# Autodesk Inventor assembly: Assembly6
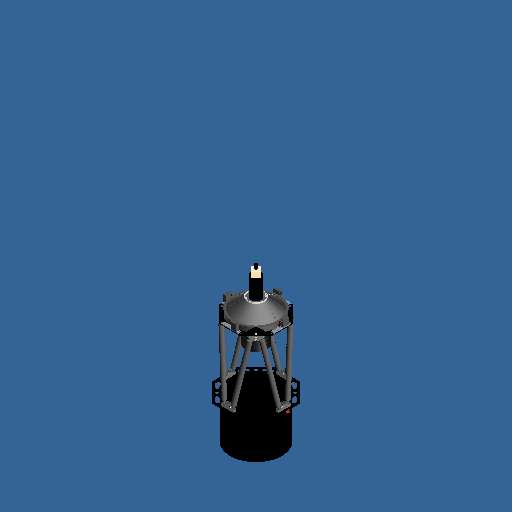
[picture p0: Inventor's stored thumbnail of the model, 512x512]
Saved by Autodesk Inventor 2026.2 (Build 302298000, 298)
## iProperties
Created: 2025-12-09
Part Number: Assembly6
Document SubType Name: Assembly
Designer: Thoma
Mass: 27295.5 g
Surface Area: 25498 cm^2
Volume: 10830.6 cm^3
Density: 2.52023 g/cm^3
Author: Thoma
## Documents named in this file (21)
- C:\Users\Thoma\OneDrive\Desktop\dir\telescope_cover\main\version_2\Main_v4.iam
- C:\Users\Thoma\OneDrive\Desktop\dir\telescope_cover\telescope\version_3\Telescope_End.ipt
- C:\Users\Thoma\OneDrive\Desktop\dir\telescope_cover\telescope\version_3\Triangle.ipt
- C:\Users\Thoma\OneDrive\Desktop\dir\telescope_cover\telescope\version_3\Triangle_Bracket_Top.ipt
- C:\Users\Thoma\OneDrive\Desktop\dir\telescope_cover\telescope\version_3\Carbon_Fibre.ipt
- C:\Users\Thoma\OneDrive\Desktop\dir\telescope_cover\telescope\version_3\5mm Screw.ipt
- C:\Users\Thoma\OneDrive\Desktop\dir\telescope_cover\telescope\version_3\35mm_bolt.ipt
- C:\Users\Thoma\OneDrive\Desktop\dir\telescope_cover\telescope\version_3\Triangle_Bracket_Bottom_MIR.ipt
- C:\Users\Thoma\OneDrive\Desktop\dir\telescope_cover\telescope\version_3\Telescope_Base.ipt
- C:\Users\Thoma\OneDrive\Desktop\dir\telescope_cover\telescope\version_3\Full_shaft_Simplify_3.ipt
- C:\Users\Thoma\OneDrive\Desktop\dir\telescope_cover\cover\Conic_Cover_Simplify_1.ipt
- C:\Users\Thoma\OneDrive\Desktop\dir\telescope_cover\telescope\version_3\30mm_bolt.ipt
- C:\Users\Thoma\OneDrive\Desktop\dir\telescope_cover\telescope\version_3\Baffle.ipt
- C:\Users\Thoma\OneDrive\Desktop\dir\telescope_cover\telescope\version_3\Bottom_End_Top.ipt
- C:\Users\Thoma\OneDrive\Desktop\dir\telescope_cover\cover\Cover_Lower_v3.ipt
- C:\Users\Thoma\OneDrive\Desktop\dir\telescope_cover\cover\Cover_Upper_v3.ipt
- C:\Users\Thoma\OneDrive\Desktop\dir\telescope_cover\telescope\version_3\4mm_0.5_Screw.ipt
- C:\Users\Thoma\OneDrive\Desktop\dir\telescope_cover\cover\Base_Plate_v2.ipt
- C:\Users\Thoma\OneDrive\Desktop\dir\telescope_cover\servo\motor_basic.ipt
- C:\Users\Thoma\OneDrive\Desktop\dir\telescope_cover\cover\rod_v6.ipt
- C:\Users\Thoma\OneDrive\Desktop\dir\telescope_cover\telescope\version_3\Laser.ipt
## Components (80 placed, 20 different names)
1. motor_basic:3 — Mate:174, Flush:138, Flush:176, Mate:175, Mate:176, Angle:85
2. motor_basic:2 — Mate:163, Flush:136, Mate:166, Mate:167, Flush:137, Angle:87
3. motor_basic:4 — Mate:191, Flush:177, Flush:178, Mate:216, Mate:219, Angle:86
4. motor_basic:5 — Mate:192, Flush:179, Flush:180, Mate:193, Mate:204, Angle:83
5. Laser:1 — Mate:215, Flush:218, Flush:219
6. Laser:2 — Mate:214, Flush:220, Flush:221
7. rod_v6:4 — Mate:216, Mate:217, Mate:218, Mate:219, Tangent:23, Angle:86
8. Full_shaft_Simplify_3:1 — Tangent:24, Tangent:25
9. Full_shaft_Simplify_3:2 — Tangent:26
10. Full_shaft_Simplify_3:3 — Tangent:27
11. Full_shaft_Simplify_3:4 — Tangent:28
12. Full_shaft_Simplify_3:5 — Tangent:29
13. Full_shaft_Simplify_3:6 — Tangent:30
14. Full_shaft_Simplify_3:7 — Tangent:32
15. Full_shaft_Simplify_3:8 — Tangent:31, Tangent:33
16. Baffle:1 — Mate:83
17. Carbon_Fibre:1 — Mate:7, Mate:11, Flush:1, Mate:12, Mate:13, Mate:14, Mate:15, Mate:62, Flush:2, Flush:3, Flush:4, Flush:5, Mate:83, Mate:92, Mate:93, Mate:96, Mate:97, Mate:98, Mate:99, Mate:100, Mate:123, Mate:124, Mate:125, Mate:213
18. Telescope_Base:1 — Mate:62, Angle:31, Mate:89, Mate:90, Angle:40, Mate:108, Mate:109, Angle:48, Mate:110, Mate:111, Angle:49, Mate:112, Mate:113, Angle:50, Mate:214, Mate:215, Flush:218, Flush:221
19. Telescope_End:1 — Mate:1, Mate:2, Angle:2, Mate:7, Mate:54, Mate:55, Angle:26, Angle:31, Mate:86, Mate:88, Mate:91, Angle:41, Mate:101, Angle:45, Angle:46, Mate:114, Mate:115, Angle:51, Mate:116, Mate:117, Angle:52, Mate:118, Mate:119, Angle:53, Mate:141, Mate:142, Mate:143, Mate:158, Mate:159, Mate:160, Mate:185, Mate:186, Mate:187, Mate:188, Mate:189, Mate:190
20. Triangle_Bracket_Top:5 — Mate:116, Mate:117, Angle:52, Mate:129, Flush:110, Angle:60
21. Triangle_Bracket_Top:4 — Mate:101, Angle:45, Angle:46, Mate:104, Mate:105, Mate:106, Flush:103, Angle:47
22. Triangle_Bracket_Top:3 — Mate:86, Mate:88, Mate:94, Angle:54, Angle:55, Mate:122, Flush:106, Angle:56
23. Triangle_Bracket_Top:1 — Mate:1, Mate:2, Angle:2, Mate:8, Mate:9, Angle:4, Mate:47, Angle:22, Mate:58
24. Triangle:1 — Mate:8, Mate:9, Angle:4, Mate:11, Flush:1, Angle:5, Angle:6, Mate:46, Mate:70, Mate:71
25. Triangle:5 — Mate:92, Mate:93, Mate:94, Mate:102, Mate:128, Flush:109, Angle:59, Mate:132, Flush:181, Angle:81
26. Triangle:6 — Mate:96, Mate:97, Mate:98, Flush:101, Angle:43, Flush:102, Angle:44, Mate:103, Mate:104, Mate:105, Mate:107
27. Triangle:7 — Mate:123, Mate:124, Mate:125, Mate:126, Flush:107, Angle:57, Mate:127, Flush:108, Angle:58, Mate:130, Mate:131
28. 35mm_bolt:6 — Mate:122, Flush:106, Angle:56
29. 35mm_bolt:7 — Mate:129, Flush:110, Angle:60
30. 35mm_bolt:4 — Mate:46, Mate:47, Angle:22
31. 35mm_bolt:5 — Mate:106, Flush:103, Angle:47
32. 5mm Screw:9 — Mate:100, Flush:102, Angle:44
33. 5mm Screw:13 — Mate:213, Flush:181, Angle:81
34. 5mm Screw:8 — Mate:99, Flush:101, Angle:43
35. 5mm Screw:10 — Mate:126, Flush:107, Angle:57
36. 5mm Screw:2 — Mate:14, Mate:15, Angle:6
37. 5mm Screw:1 — Mate:12, Mate:13, Angle:5
38. 5mm Screw:11 — Mate:127, Flush:108, Angle:58
39. 5mm Screw:12 — Mate:128, Flush:109, Angle:59
40. 30mm_bolt:7 — Mate:120, Flush:104, Angle:54
41. 30mm_bolt:1 — Mate:121, Flush:105, Angle:55
42. 30mm_bolt:8 — Mate:80, Flush:13, Angle:39
43. 30mm_bolt:6 — Mate:78, Flush:11, Angle:37
44. 30mm_bolt:3 — Mate:79, Flush:12, Angle:38
45. 30mm_bolt:2 — Mate:77, Flush:10, Angle:36
46. Triangle_Bracket_Bottom_MIR:4 — Mate:118, Mate:119, Angle:53, Tangent:24
47. Triangle_Bracket_Bottom_MIR:3 — Mate:114, Mate:115, Angle:51, Mate:120, Flush:104, Mate:121, Flush:105, Tangent:27, Tangent:28
48. Triangle_Bracket_Bottom_MIR:2 — Mate:55, Mate:58, Angle:26, Mate:77, Flush:10, Angle:36, Mate:78, Flush:11, Angle:37, Tangent:30, Tangent:31
49. Triangle_Bracket_Bottom_MIR:1 — Mate:54, Mate:79, Flush:12, Angle:38, Mate:80, Flush:13, Angle:39, Mate:91, Angle:41, Tangent:29, Tangent:32
50. Bottom_End_Top:4 — Mate:112, Mate:113, Angle:50, Tangent:26, Tangent:33
51. Bottom_End_Top:3 — Mate:110, Mate:111, Angle:49, Flush:219, Tangent:25
52. Bottom_End_Top:2 — Mate:108, Mate:109, Angle:48
53. Bottom_End_Top:1 — Mate:89, Mate:90, Angle:40, Flush:220
54. Conic_Cover_Simplify_1:1 — Flush:2, Mate:131, Mate:132
55. Conic_Cover_Simplify_1:2 — Flush:3, Mate:102, Mate:103
56. Conic_Cover_Simplify_1:3 — Flush:4, Mate:70, Mate:107
57. Conic_Cover_Simplify_1:4 — Mate:71, Flush:5, Mate:130
58. Cover_Lower_v3:2 — Tangent:22, Mate:205, Mate:206, Mate:207, Mate:208, Mate:209, Mate:210, Mate:211, Mate:212
59. 4mm_0.5_Screw:15 — Mate:211, Mate:212, Angle:79
60. 4mm_0.5_Screw:14 — Mate:209, Mate:210, Angle:78, Angle:79
61. 4mm_0.5_Screw:13 — Mate:207, Mate:208, Angle:77, Angle:78
62. rod_v6:3 — Mate:193, Mate:204, Tangent:22, Mate:205, Mate:206, Angle:77, Angle:83
63. Base_Plate_v2:4 — Mate:188, Mate:189, Mate:190, Mate:192, Flush:179, Flush:180
64. 4mm_0.5_Screw:10 — Mate:198, Mate:199, Mate:217
65. 4mm_0.5_Screw:11 — Mate:200, Mate:201, Angle:76
66. 4mm_0.5_Screw:12 — Mate:202, Mate:203, Angle:76, Mate:218
67. Cover_Upper_v3:2 — Mate:198, Mate:199, Mate:200, Mate:201, Mate:202, Mate:203, Tangent:23
68. Base_Plate_v2:3 — Mate:185, Mate:186, Mate:187, Mate:191, Flush:177, Flush:178
69. 4mm_0.5_Screw:9 — Mate:183, Mate:184, Angle:73
70. 4mm_0.5_Screw:8 — Mate:181, Mate:182, Angle:72, Angle:73
71. 4mm_0.5_Screw:7 — Mate:179, Mate:180, Angle:71, Angle:72
72. rod_v6:2 — Mate:175, Mate:176, Mate:177, Mate:178, Tangent:20, Angle:71, Angle:85
73. Cover_Lower_v3:1 — Mate:177, Mate:178, Tangent:20, Mate:179, Mate:180, Mate:181, Mate:182, Mate:183, Mate:184
74. 4mm_0.5_Screw:6 — Mate:168, Mate:169, Angle:68, Angle:69
75. 4mm_0.5_Screw:5 — Mate:170, Mate:171, Angle:69, Angle:70
76. 4mm_0.5_Screw:4 — Mate:172, Mate:173, Angle:70
77. rod_v6:1 — Mate:164, Mate:165, Tangent:19, Mate:166, Mate:167, Angle:68, Angle:87
78. Cover_Upper_v3:1 — Mate:164, Mate:165, Tangent:19, Mate:168, Mate:169, Mate:170, Mate:171, Mate:172, Mate:173
79. Base_Plate_v2:2 — Mate:158, Mate:159, Mate:160, Mate:163, Flush:136, Flush:137
80. Base_Plate_v2:1 — Mate:141, Mate:142, Mate:143, Mate:174, Flush:138, Flush:176
## Relationships (219: Mate 127, Angle 46, Flush 32, Tangent 14)
- Mate:1: Telescope_End:1 ↔ Triangle_Bracket_Top:1
- Mate:2: Telescope_End:1 ↔ Triangle_Bracket_Top:1
- Angle:2 (0 deg): Telescope_End:1 ↔ Triangle_Bracket_Top:1
- Mate:7: Carbon_Fibre:1 ↔ Telescope_End:1
- Mate:8: Triangle_Bracket_Top:1 ↔ Triangle:1
- Mate:9: Triangle_Bracket_Top:1 ↔ Triangle:1
- Angle:4 (0 deg): Triangle_Bracket_Top:1 ↔ Triangle:1
- Mate:11: Carbon_Fibre:1 ↔ Triangle:1
- Flush:1: Carbon_Fibre:1 ↔ Triangle:1
- Mate:12: Carbon_Fibre:1 ↔ 5mm Screw:1
- Mate:13: Carbon_Fibre:1 ↔ 5mm Screw:1
- Angle:5 (0 deg): Triangle:1 ↔ 5mm Screw:1
- Mate:14: Carbon_Fibre:1 ↔ 5mm Screw:2
- Mate:15: Carbon_Fibre:1 ↔ 5mm Screw:2
- Angle:6 (0 deg): Triangle:1 ↔ 5mm Screw:2
- Mate:46: Triangle:1 ↔ 35mm_bolt:4
- Mate:47: Triangle_Bracket_Top:1 ↔ 35mm_bolt:4
- Angle:22 (0 deg): Triangle_Bracket_Top:1 ↔ 35mm_bolt:4
- Mate:54: Telescope_End:1 ↔ Triangle_Bracket_Bottom_MIR:1
- Mate:55: Telescope_End:1 ↔ Triangle_Bracket_Bottom_MIR:2
- Mate:58: Triangle_Bracket_Top:1 ↔ Triangle_Bracket_Bottom_MIR:2
- Angle:26 (0 deg): Telescope_End:1 ↔ Triangle_Bracket_Bottom_MIR:2
- Mate:62: Carbon_Fibre:1 ↔ Telescope_Base:1
- Angle:31 (0 deg): Telescope_Base:1 ↔ Telescope_End:1
- Flush:2: Carbon_Fibre:1 ↔ Conic_Cover_Simplify_1:1
- Flush:3: Carbon_Fibre:1 ↔ Conic_Cover_Simplify_1:2
- Flush:4: Carbon_Fibre:1 ↔ Conic_Cover_Simplify_1:3
- Mate:70: Triangle:1 ↔ Conic_Cover_Simplify_1:3
- Mate:71: Triangle:1 ↔ Conic_Cover_Simplify_1:4
- Flush:5: Carbon_Fibre:1 ↔ Conic_Cover_Simplify_1:4
- Mate:77: 30mm_bolt:2 ↔ Triangle_Bracket_Bottom_MIR:2
- Flush:10: 30mm_bolt:2 ↔ Triangle_Bracket_Bottom_MIR:2
- Angle:36 (0 deg): 30mm_bolt:2 ↔ Triangle_Bracket_Bottom_MIR:2
- Mate:78: 30mm_bolt:6 ↔ Triangle_Bracket_Bottom_MIR:2
- Flush:11: 30mm_bolt:6 ↔ Triangle_Bracket_Bottom_MIR:2
- Angle:37 (0 deg): 30mm_bolt:6 ↔ Triangle_Bracket_Bottom_MIR:2
- Mate:79: 30mm_bolt:3 ↔ Triangle_Bracket_Bottom_MIR:1
- Flush:12: 30mm_bolt:3 ↔ Triangle_Bracket_Bottom_MIR:1
- Angle:38 (0 deg): 30mm_bolt:3 ↔ Triangle_Bracket_Bottom_MIR:1
- Mate:80: 30mm_bolt:8 ↔ Triangle_Bracket_Bottom_MIR:1
- Flush:13: 30mm_bolt:8 ↔ Triangle_Bracket_Bottom_MIR:1
- Angle:39 (0 deg): 30mm_bolt:8 ↔ Triangle_Bracket_Bottom_MIR:1
- Mate:83: Baffle:1 ↔ Carbon_Fibre:1
- Mate:86: Telescope_End:1 ↔ Triangle_Bracket_Top:3
- Mate:88: Telescope_End:1 ↔ Triangle_Bracket_Top:3
- Mate:89: Telescope_Base:1 ↔ Bottom_End_Top:1
- Mate:90: Telescope_Base:1 ↔ Bottom_End_Top:1
- Angle:40 (0 deg): Telescope_Base:1 ↔ Bottom_End_Top:1
- Mate:91: Telescope_End:1 ↔ Triangle_Bracket_Bottom_MIR:1
- Angle:41 (0 deg): Telescope_End:1 ↔ Triangle_Bracket_Bottom_MIR:1
- Mate:92: Carbon_Fibre:1 ↔ Triangle:5
- Mate:93: Carbon_Fibre:1 ↔ Triangle:5
- Mate:94: Triangle_Bracket_Top:3 ↔ Triangle:5
- Mate:96: Carbon_Fibre:1 ↔ Triangle:6
- Mate:97: Carbon_Fibre:1 ↔ Triangle:6
- Mate:98: Carbon_Fibre:1 ↔ Triangle:6
- Mate:99: Carbon_Fibre:1 ↔ 5mm Screw:8
- Flush:101: Triangle:6 ↔ 5mm Screw:8
- Angle:43 (0 deg): Triangle:6 ↔ 5mm Screw:8
- Mate:100: Carbon_Fibre:1 ↔ 5mm Screw:9
- Flush:102: Triangle:6 ↔ 5mm Screw:9
- Angle:44 (0 deg): Triangle:6 ↔ 5mm Screw:9
- Mate:101: Telescope_End:1 ↔ Triangle_Bracket_Top:4
- Angle:45 (0 deg): Telescope_End:1 ↔ Triangle_Bracket_Top:4
- Mate:102: Triangle:5 ↔ Conic_Cover_Simplify_1:2
- Mate:103: Triangle:6 ↔ Conic_Cover_Simplify_1:2
- Angle:46 (0 deg): Telescope_End:1 ↔ Triangle_Bracket_Top:4
- Mate:104: Triangle_Bracket_Top:4 ↔ Triangle:6
- Mate:105: Triangle_Bracket_Top:4 ↔ Triangle:6
- Mate:106: Triangle_Bracket_Top:4 ↔ 35mm_bolt:5
- Flush:103: Triangle_Bracket_Top:4 ↔ 35mm_bolt:5
- Angle:47 (0 deg): Triangle_Bracket_Top:4 ↔ 35mm_bolt:5
- Mate:107: Triangle:6 ↔ Conic_Cover_Simplify_1:3
- Mate:108: Telescope_Base:1 ↔ Bottom_End_Top:2
- Mate:109: Telescope_Base:1 ↔ Bottom_End_Top:2
- Angle:48 (0 deg): Telescope_Base:1 ↔ Bottom_End_Top:2
- Mate:110: Telescope_Base:1 ↔ Bottom_End_Top:3
- Mate:111: Telescope_Base:1 ↔ Bottom_End_Top:3
- Angle:49 (0 deg): Telescope_Base:1 ↔ Bottom_End_Top:3
- Mate:112: Telescope_Base:1 ↔ Bottom_End_Top:4
- Mate:113: Telescope_Base:1 ↔ Bottom_End_Top:4
- Angle:50 (0 deg): Telescope_Base:1 ↔ Bottom_End_Top:4
- Mate:114: Telescope_End:1 ↔ Triangle_Bracket_Bottom_MIR:3
- Mate:115: Telescope_End:1 ↔ Triangle_Bracket_Bottom_MIR:3
- Angle:51 (0 deg): Telescope_End:1 ↔ Triangle_Bracket_Bottom_MIR:3
- Mate:116: Telescope_End:1 ↔ Triangle_Bracket_Top:5
- Mate:117: Telescope_End:1 ↔ Triangle_Bracket_Top:5
- Angle:52 (0 deg): Telescope_End:1 ↔ Triangle_Bracket_Top:5
- Mate:118: Telescope_End:1 ↔ Triangle_Bracket_Bottom_MIR:4
- Mate:119: Telescope_End:1 ↔ Triangle_Bracket_Bottom_MIR:4
- Angle:53 (0 deg): Telescope_End:1 ↔ Triangle_Bracket_Bottom_MIR:4
- Mate:120: 30mm_bolt:7 ↔ Triangle_Bracket_Bottom_MIR:3
- Flush:104: 30mm_bolt:7 ↔ Triangle_Bracket_Bottom_MIR:3
- Angle:54 (0 deg): Triangle_Bracket_Top:3 ↔ 30mm_bolt:7
- Mate:121: 30mm_bolt:1 ↔ Triangle_Bracket_Bottom_MIR:3
- Flush:105: 30mm_bolt:1 ↔ Triangle_Bracket_Bottom_MIR:3
- Angle:55 (0 deg): Triangle_Bracket_Top:3 ↔ 30mm_bolt:1
- Mate:122: Triangle_Bracket_Top:3 ↔ 35mm_bolt:6
- Flush:106: Triangle_Bracket_Top:3 ↔ 35mm_bolt:6
- Angle:56 (0 deg): Triangle_Bracket_Top:3 ↔ 35mm_bolt:6
- Mate:123: Carbon_Fibre:1 ↔ Triangle:7
- Mate:124: Carbon_Fibre:1 ↔ Triangle:7
- Mate:125: Carbon_Fibre:1 ↔ Triangle:7
- Mate:126: Triangle:7 ↔ 5mm Screw:10
- Flush:107: Triangle:7 ↔ 5mm Screw:10
- Angle:57 (0 deg): Triangle:7 ↔ 5mm Screw:10
- Mate:127: Triangle:7 ↔ 5mm Screw:11
- Flush:108: Triangle:7 ↔ 5mm Screw:11
- Angle:58 (0 deg): Triangle:7 ↔ 5mm Screw:11
- Mate:128: Triangle:5 ↔ 5mm Screw:12
- Flush:109: Triangle:5 ↔ 5mm Screw:12
- Angle:59 (0 deg): Triangle:5 ↔ 5mm Screw:12
- Mate:129: Triangle_Bracket_Top:5 ↔ 35mm_bolt:7
- Flush:110: Triangle_Bracket_Top:5 ↔ 35mm_bolt:7
- Angle:60 (0 deg): Triangle_Bracket_Top:5 ↔ 35mm_bolt:7
- Mate:130: Triangle:7 ↔ Conic_Cover_Simplify_1:4
- Mate:131: Triangle:7 ↔ Conic_Cover_Simplify_1:1
- Mate:132: Triangle:5 ↔ Conic_Cover_Simplify_1:1
- Mate:141: Telescope_End:1 ↔ Base_Plate_v2:1
- Mate:142: Telescope_End:1 ↔ Base_Plate_v2:1
- Mate:143: Telescope_End:1 ↔ Base_Plate_v2:1
- Mate:158: Telescope_End:1 ↔ Base_Plate_v2:2
- Mate:159: Telescope_End:1 ↔ Base_Plate_v2:2
- Mate:160: Telescope_End:1 ↔ Base_Plate_v2:2
- Mate:163: motor_basic:2 ↔ Base_Plate_v2:2
- Flush:136: motor_basic:2 ↔ Base_Plate_v2:2
- Mate:164: rod_v6:1 ↔ Cover_Upper_v3:1
- Mate:165: rod_v6:1 ↔ Cover_Upper_v3:1
- Tangent:19 (-1 mm): rod_v6:1 ↔ Cover_Upper_v3:1
- Mate:166: motor_basic:2 ↔ rod_v6:1
- Mate:167 (2 mm): motor_basic:2 ↔ rod_v6:1
- Mate:168: 4mm_0.5_Screw:6 ↔ Cover_Upper_v3:1
- Mate:169: 4mm_0.5_Screw:6 ↔ Cover_Upper_v3:1
- Angle:68 (0 deg): 4mm_0.5_Screw:6 ↔ rod_v6:1
- Mate:170: 4mm_0.5_Screw:5 ↔ Cover_Upper_v3:1
- Mate:171: 4mm_0.5_Screw:5 ↔ Cover_Upper_v3:1
- Angle:69 (0 deg): 4mm_0.5_Screw:6 ↔ 4mm_0.5_Screw:5
- Mate:172: 4mm_0.5_Screw:4 ↔ Cover_Upper_v3:1
- Mate:173: 4mm_0.5_Screw:4 ↔ Cover_Upper_v3:1
- Angle:70 (0 deg): 4mm_0.5_Screw:5 ↔ 4mm_0.5_Screw:4
- Flush:137 (13.495 mm): motor_basic:2 ↔ Base_Plate_v2:2
- Mate:174: motor_basic:3 ↔ Base_Plate_v2:1
- Flush:138: motor_basic:3 ↔ Base_Plate_v2:1
- Flush:176 (13.495 mm): motor_basic:3 ↔ Base_Plate_v2:1
- Mate:175: motor_basic:3 ↔ rod_v6:2
- Mate:176 (2 mm): motor_basic:3 ↔ rod_v6:2
- Mate:177: rod_v6:2 ↔ Cover_Lower_v3:1
- Mate:178: rod_v6:2 ↔ Cover_Lower_v3:1
- Tangent:20 (-1 mm): rod_v6:2 ↔ Cover_Lower_v3:1
- Mate:179: 4mm_0.5_Screw:7 ↔ Cover_Lower_v3:1
- Mate:180: 4mm_0.5_Screw:7 ↔ Cover_Lower_v3:1
- Angle:71 (0 deg): 4mm_0.5_Screw:7 ↔ rod_v6:2
- Mate:181: 4mm_0.5_Screw:8 ↔ Cover_Lower_v3:1
- Mate:182: 4mm_0.5_Screw:8 ↔ Cover_Lower_v3:1
- Angle:72 (0 deg): 4mm_0.5_Screw:8 ↔ 4mm_0.5_Screw:7
- Mate:183: 4mm_0.5_Screw:9 ↔ Cover_Lower_v3:1
- Mate:184: 4mm_0.5_Screw:9 ↔ Cover_Lower_v3:1
- Angle:73 (0 deg): 4mm_0.5_Screw:9 ↔ 4mm_0.5_Screw:8
- Mate:185: Telescope_End:1 ↔ Base_Plate_v2:3
- Mate:186: Telescope_End:1 ↔ Base_Plate_v2:3
- Mate:187: Telescope_End:1 ↔ Base_Plate_v2:3
- Mate:188: Telescope_End:1 ↔ Base_Plate_v2:4
- Mate:189: Telescope_End:1 ↔ Base_Plate_v2:4
- Mate:190: Telescope_End:1 ↔ Base_Plate_v2:4
- Mate:191: motor_basic:4 ↔ Base_Plate_v2:3
- Flush:177: motor_basic:4 ↔ Base_Plate_v2:3
- Flush:178 (13.495 mm): motor_basic:4 ↔ Base_Plate_v2:3
- Mate:192: motor_basic:5 ↔ Base_Plate_v2:4
- Flush:179: motor_basic:5 ↔ Base_Plate_v2:4
- Flush:180 (13.495 mm): motor_basic:5 ↔ Base_Plate_v2:4
- Mate:193: motor_basic:5 ↔ rod_v6:3
- Mate:198: 4mm_0.5_Screw:10 ↔ Cover_Upper_v3:2
- Mate:199: 4mm_0.5_Screw:10 ↔ Cover_Upper_v3:2
- Mate:200: 4mm_0.5_Screw:11 ↔ Cover_Upper_v3:2
- Mate:201: 4mm_0.5_Screw:11 ↔ Cover_Upper_v3:2
- Mate:202: 4mm_0.5_Screw:12 ↔ Cover_Upper_v3:2
- Mate:203: 4mm_0.5_Screw:12 ↔ Cover_Upper_v3:2
- Angle:76 (0 deg): 4mm_0.5_Screw:11 ↔ 4mm_0.5_Screw:12
- Mate:204 (2 mm): motor_basic:5 ↔ rod_v6:3
- Tangent:22 (-1 mm): Cover_Lower_v3:2 ↔ rod_v6:3
- Mate:205: Cover_Lower_v3:2 ↔ rod_v6:3
- Mate:206: Cover_Lower_v3:2 ↔ rod_v6:3
- Mate:207: Cover_Lower_v3:2 ↔ 4mm_0.5_Screw:13
- Mate:208: Cover_Lower_v3:2 ↔ 4mm_0.5_Screw:13
- Angle:77 (0 deg): 4mm_0.5_Screw:13 ↔ rod_v6:3
- Mate:209: Cover_Lower_v3:2 ↔ 4mm_0.5_Screw:14
- Mate:210: Cover_Lower_v3:2 ↔ 4mm_0.5_Screw:14
- Angle:78 (0 deg): 4mm_0.5_Screw:14 ↔ 4mm_0.5_Screw:13
- Mate:211: Cover_Lower_v3:2 ↔ 4mm_0.5_Screw:15
- Mate:212: Cover_Lower_v3:2 ↔ 4mm_0.5_Screw:15
- Angle:79 (0 deg): 4mm_0.5_Screw:15 ↔ 4mm_0.5_Screw:14
- Mate:213: Carbon_Fibre:1 ↔ 5mm Screw:13
- Flush:181: Triangle:5 ↔ 5mm Screw:13
- Angle:81 (0 deg): Triangle:5 ↔ 5mm Screw:13
- Mate:214: Laser:2 ↔ Telescope_Base:1
- Mate:215: Laser:1 ↔ Telescope_Base:1
- Flush:218: Laser:1 ↔ Telescope_Base:1
- Flush:219 (39.316 mm): Laser:1 ↔ Bottom_End_Top:3
- Flush:220 (39.316 mm): Laser:2 ↔ Bottom_End_Top:1
- Flush:221: Laser:2 ↔ Telescope_Base:1
- Mate:216: motor_basic:4 ↔ rod_v6:4
- Mate:217: rod_v6:4 ↔ 4mm_0.5_Screw:10
- Mate:218: rod_v6:4 ↔ 4mm_0.5_Screw:12
- Mate:219 (2 mm): motor_basic:4 ↔ rod_v6:4
- Tangent:23 (-1 mm): rod_v6:4 ↔ Cover_Upper_v3:2
- Angle:83 (9.573 deg): motor_basic:5 ↔ rod_v6:3
- Angle:85 (9.573 deg): motor_basic:3 ↔ rod_v6:2
- Angle:86 (9.573 deg): motor_basic:4 ↔ rod_v6:4
- Angle:87 (9.573 deg): motor_basic:2 ↔ rod_v6:1
- Tangent:24: Full_shaft_Simplify_3:1 ↔ Triangle_Bracket_Bottom_MIR:4
- Tangent:25: Full_shaft_Simplify_3:1 ↔ Bottom_End_Top:3
- Tangent:26: Full_shaft_Simplify_3:2 ↔ Bottom_End_Top:4
- Tangent:27: Full_shaft_Simplify_3:3 ↔ Triangle_Bracket_Bottom_MIR:3
- Tangent:28: Full_shaft_Simplify_3:4 ↔ Triangle_Bracket_Bottom_MIR:3
- Tangent:29: Full_shaft_Simplify_3:5 ↔ Triangle_Bracket_Bottom_MIR:1
- Tangent:30: Full_shaft_Simplify_3:6 ↔ Triangle_Bracket_Bottom_MIR:2
- Tangent:31: Full_shaft_Simplify_3:8 ↔ Triangle_Bracket_Bottom_MIR:2
- Tangent:32: Full_shaft_Simplify_3:7 ↔ Triangle_Bracket_Bottom_MIR:1
- Tangent:33: Full_shaft_Simplify_3:8 ↔ Bottom_End_Top:4
